# Autodesk Inventor assembly: zmotorblock
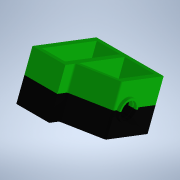
[picture p0: Inventor's stored thumbnail of the model, 180x180]
Saved by Autodesk Inventor 2020.4 (Build 244396000, 396)
## iProperties
Created: 2021-03-29
Part Number: zmotorblock
Document SubType Name: Assembly
Designer: AOB
Mass: 82.5513 g
Surface Area: 367.693 cm^2
Volume: 77.8786 cm^3
Density: 1.06 g/cm^3
Author: AOB
## Documents named in this file (3)
- C:\Users\marti\Documents\Inventor\ProjectBoron\Boron Ultima\zmotorblock.iam
- C:\Users\marti\Documents\Inventor\ProjectBoron\Boron Ultima\zmotorblockleft-half.ipt
- C:\Users\marti\Documents\Inventor\ProjectBoron\Boron Ultima\zmotorblockright-half.ipt
## Components (2 placed, 2 different names)
1. zmotorblockleft-half:1 — Rigid:1
2. zmotorblockright-half:1 — Rigid:1
## Relationships (1: WeldJoint 1)
- Rigid:1 [WeldJoint]: zmotorblockleft-half:1 ↔ zmotorblockright-half:1
